# Autodesk Inventor assembly: aftServoSectionAssembly0
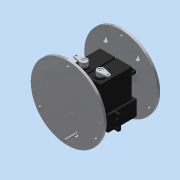
[picture p0: Inventor's stored thumbnail of the model, 180x180]
Saved by Autodesk Inventor 2017 (Build 210142000, 142)
## iProperties
Created: 2016-10-29
Part Number: aftServoSectionAssembly0
Document SubType Name: Assembly
Designer: techn
Author: techn
## Documents named in this file (6)
- D:\OneDrive\Documents\Other Projects\Submarine\CAD\midships\AftServoSection\aftServoSectionAssembly0.iam
- D:\OneDrive\Documents\Other Projects\Submarine\CAD\midships\AftServoSection\rearServoAttachmentPlate.ipt
- D:\OneDrive\Documents\Other Projects\Submarine\CAD\common\HitecServo\HitecServoAssembly.iam
- D:\OneDrive\Documents\Other Projects\Submarine\CAD\midships\AftServoSection\frontServoAttachmentPlate.ipt
- D:\OneDrive\Documents\Other Projects\Submarine\CAD\common\HitecServo\ServoHorn10mmPitch.ipt
- D:\OneDrive\Documents\Other Projects\Submarine\CAD\common\3mmShaftToServo\ServoWithShaftAssembly.iam
## Components (7 placed, 5 different names)
1. rearServoAttachmentPlate:1 — Mate:1, Mate:2, Mate:3, Mate:4, Mate:5, Mate:6, Mate:17, Flush:1
2. HitecServoAssembly:1 [sub-assembly] — Mate:2, Mate:3, Mate:6, Mate:10, Mate:11, Mate:13, Mate:14, Mate:16
3. HitecServoAssembly:2 [sub-assembly] — Mate:1, Mate:4, Mate:5, Mate:9, Mate:12, Mate:15
4. frontServoAttachmentPlate:1 — Mate:9, Mate:10, Mate:11
5. ServoHorn10mmPitch:1 — Mate:13, Mate:14
6. ServoHorn10mmPitch:2 — Mate:12, Mate:15
7. ServoWithShaftAssembly:1 [sub-assembly] — Mate:16, Mate:17, Flush:1
## Relationships (16: Mate 15, Flush 1)
- Mate:1: rearServoAttachmentPlate:1 ↔ HitecServoAssembly:2
- Mate:2: rearServoAttachmentPlate:1 ↔ HitecServoAssembly:1
- Mate:3: rearServoAttachmentPlate:1 ↔ HitecServoAssembly:1
- Mate:4: rearServoAttachmentPlate:1 ↔ HitecServoAssembly:2
- Mate:5: rearServoAttachmentPlate:1 ↔ HitecServoAssembly:2
- Mate:6: rearServoAttachmentPlate:1 ↔ HitecServoAssembly:1
- Mate:9: HitecServoAssembly:2 ↔ frontServoAttachmentPlate:1
- Mate:10: HitecServoAssembly:1 ↔ frontServoAttachmentPlate:1
- Mate:11: HitecServoAssembly:1 ↔ frontServoAttachmentPlate:1
- Mate:12: HitecServoAssembly:2 ↔ ServoHorn10mmPitch:2
- Mate:13: HitecServoAssembly:1 ↔ ServoHorn10mmPitch:1
- Mate:14: HitecServoAssembly:1 ↔ ServoHorn10mmPitch:1
- Mate:15: HitecServoAssembly:2 ↔ ServoHorn10mmPitch:2
- Mate:16 (2.54 mm): HitecServoAssembly:1 ↔ ServoWithShaftAssembly:1
- Mate:17: rearServoAttachmentPlate:1 ↔ ServoWithShaftAssembly:1
- Flush:1 (-28.194 mm): rearServoAttachmentPlate:1 ↔ ServoWithShaftAssembly:1
